# Autodesk Inventor assembly: SGB-assembly
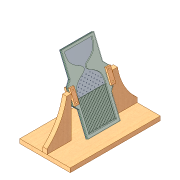
[picture p0: Inventor's stored thumbnail of the model, 180x180]
Saved by Autodesk Inventor 2020 (Build 240168000, 168)
## iProperties
Created: 2021-06-24
Part Number: SGB-assembly
Document SubType Name: Assembly
Designer: Aidan Lee
Author: Aidan Lee
## Documents named in this file (9)
- C:\Users\hobly\OneDrive\0_UCD-Internship\Upload2Dropbox\GaltonBoard\SGB-assembly.iam
- C:\Users\hobly\OneDrive\0_UCD-Internship\Upload2Dropbox\GaltonBoard\SGB-1-front.ipt
- C:\Users\hobly\OneDrive\0_UCD-Internship\Upload2Dropbox\GaltonBoard\SGB-2-middle.ipt
- C:\Users\hobly\OneDrive\0_UCD-Internship\Upload2Dropbox\GaltonBoard\SGB-3-bins.ipt
- C:\Users\hobly\OneDrive\0_UCD-Internship\Upload2Dropbox\GaltonBoard\SGB-4-back.ipt
- C:\Users\hobly\OneDrive\0_UCD-Internship\Upload2Dropbox\GaltonBoard\SGB-5-backcover.ipt
- C:\Users\hobly\OneDrive\0_UCD-Internship\Upload2Dropbox\GaltonBoard\SGB-6-hinge.ipt
- C:\Users\hobly\OneDrive\0_UCD-Internship\Upload2Dropbox\GaltonBoard\SGB-7-arm.ipt
- C:\Users\hobly\OneDrive\0_UCD-Internship\Upload2Dropbox\GaltonBoard\SGB-8-platform.ipt
## Components (10 placed, 8 different names)
1. SGB-1-front:1 — Flush:4, Flush:5, Mate:4, Mate:12
2. SGB-2-middle:1 — Mate:1, Flush:1, Flush:2, Mate:2, Mate:3, Flush:3, Flush:4, Flush:5, Mate:4, Mate:7, Mate:8, Mate:10, Mate:11, Mate:14
3. SGB-3-bins:1 — Mate:2, Mate:3, Flush:3
4. SGB-4-back:1 — Mate:1, Flush:1, Flush:2, Mate:5, Flush:6, Mate:6, Mate:9
5. SGB-5-backcover:1 — Mate:5, Flush:6, Mate:6
6. SGB-6-hinge:1 — Mate:7, Mate:8, Mate:9, Mate:15, Mate:16
7. SGB-7-arm:1 — Mate:13, Mate:14, Mate:18
8. SGB-8-platform:1 — Mate:17, Mate:18, Mate:19
9. SGB-6-hinge:2 — Mate:10, Mate:11, Mate:12, Mate:13
10. SGB-7-arm:2 — Mate:15, Mate:16, Mate:17, Mate:19
## Relationships (25: Mate 19, Flush 6)
- Mate:1: SGB-2-middle:1 ↔ SGB-4-back:1
- Flush:1: SGB-2-middle:1 ↔ SGB-4-back:1
- Flush:2: SGB-2-middle:1 ↔ SGB-4-back:1
- Mate:2: SGB-2-middle:1 ↔ SGB-3-bins:1
- Mate:3: SGB-2-middle:1 ↔ SGB-3-bins:1
- Flush:3: SGB-2-middle:1 ↔ SGB-3-bins:1
- Flush:4: SGB-1-front:1 ↔ SGB-2-middle:1
- Flush:5: SGB-1-front:1 ↔ SGB-2-middle:1
- Mate:4: SGB-1-front:1 ↔ SGB-2-middle:1
- Mate:5: SGB-4-back:1 ↔ SGB-5-backcover:1
- Flush:6: SGB-4-back:1 ↔ SGB-5-backcover:1
- Mate:6 (-11.45 mm): SGB-4-back:1 ↔ SGB-5-backcover:1
- Mate:7: SGB-2-middle:1 ↔ SGB-6-hinge:1
- Mate:8: SGB-2-middle:1 ↔ SGB-6-hinge:1
- Mate:9: SGB-4-back:1 ↔ SGB-6-hinge:1
- Mate:10: SGB-2-middle:1 ↔ SGB-6-hinge:2
- Mate:11: SGB-2-middle:1 ↔ SGB-6-hinge:2
- Mate:12: SGB-1-front:1 ↔ SGB-6-hinge:2
- Mate:13: SGB-7-arm:1 ↔ SGB-6-hinge:2
- Mate:14 (2.1 mm): SGB-2-middle:1 ↔ SGB-7-arm:1
- Mate:15 (2.1 mm): SGB-6-hinge:1 ↔ SGB-7-arm:2
- Mate:16: SGB-6-hinge:1 ↔ SGB-7-arm:2
- Mate:17: SGB-8-platform:1 ↔ SGB-7-arm:2
- Mate:18: SGB-7-arm:1 ↔ SGB-8-platform:1
- Mate:19: SGB-8-platform:1 ↔ SGB-7-arm:2
